# Autodesk Inventor assembly: Ensamble
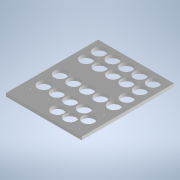
[picture p0: Inventor's stored thumbnail of the model, 180x180]
Saved by Autodesk Inventor 2020.3 (Build 243373000, 373)
## iProperties
Created: 2021-04-10
Part Number: Ensamble
Document SubType Name: Assembly
Designer: juanp
Author: juanp
## Documents named in this file (3)
- C:\Users\juanp\Desktop\Files - Temp\Cajas Electronica\Ensamble.iam
- C:\Users\juanp\Desktop\Files - Temp\Cajas Electronica\Conectores2.ipt
- C:\Users\juanp\Desktop\Files - Temp\Cajas Electronica\Conectores1.ipt
## Components (2 placed, 2 different names)
1. Conectores2:1 — Flush:1, Flush:2, Mate:1, Flush:3
2. Conectores1:1 — Flush:1, Flush:2, Mate:1, Flush:3
## Relationships (4: Flush 3, Mate 1)
- Flush:1: Conectores2:1 ↔ Conectores1:1
- Flush:2: Conectores2:1 ↔ Conectores1:1
- Mate:1: Conectores2:1 ↔ Conectores1:1
- Flush:3: Conectores2:1 ↔ Conectores1:1
